# Autodesk Inventor assembly: ESP32ParasiteMicroscope_v0
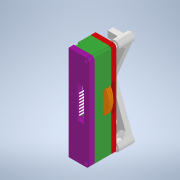
[picture p0: Inventor's stored thumbnail of the model, 180x180]
Saved by Autodesk Inventor 2022 (Build 260153000, 153)
## iProperties
Created: 2022-02-01
Part Number: ESP32ParasiteMicroscope_v0
Document SubType Name: Assembly
Designer: diederichbenedict
Author: diederichbenedict
## Documents named in this file (9)
- C:\Users\Prakash Lab\Documents\Matchboxscope\INVENTOR\ESP32ParasiteMicroscope_v0.iam
- C:\Users\Prakash Lab\Documents\Matchboxscope\INVENTOR\00_chip.ipt
- C:\Users\Prakash Lab\Documents\Matchboxscope\INVENTOR\00_ESP3-CAM.iam
- C:\Users\Prakash Lab\Documents\Matchboxscope\INVENTOR\ESP32ParasiteMicroscope_base_v0.ipt
- C:\Users\Prakash Lab\Documents\Matchboxscope\INVENTOR\ESP32ParasiteMicroscope_top_v0.ipt
- C:\Users\Prakash Lab\Documents\Matchboxscope\INVENTOR\ESP32ParasiteMicroscope_lid_v0.ipt
- C:\Users\diederichbenedict\Documents\Inventor\Content Center Files\R2022\de-DE\DIN 912\DIN 912 - M3 x 0.5 x 25 x 18.ipt
- C:\Users\Prakash Lab\Documents\Matchboxscope\INVENTOR\ESP32ParasiteMicroscope_middle_v1.ipt
- C:\Users\Prakash Lab\Documents\Matchboxscope\INVENTOR\ESP32ParasiteMicroscope_focusknob_v1.ipt
## Components (12 placed, 8 different names)
1. 00_chip:1
2. ESP32ParasiteMicroscope_base_v0:1 — Fluchtend:3, Fluchtend:4
3. ESP32ParasiteMicroscope_middle_v1:1 — Fluchtend:3, Fluchtend:4, Fluchtend:5, Fluchtend:6, Fluchtend:8, Fluchtend:9
4. ESP32ParasiteMicroscope_focusknob_v1:1 — Fluchtend:5, Fluchtend:6, Passend:1
5. ESP32ParasiteMicroscope_top_v0:1 — Fluchtend:8, Fluchtend:9, Fluchtend:10, Fluchtend:11
6. ESP32ParasiteMicroscope_lid_v0:1 — Fluchtend:10, Fluchtend:11, Einfügen:6
7. DIN 912 - ersetzt durch DIN EN ISO 4762 M3 x 25:1
8. DIN 912 - ersetzt durch DIN EN ISO 4762 M3 x 25:2
9. DIN 912 - ersetzt durch DIN EN ISO 4762 M3 x 25:3
10. DIN 912 - ersetzt durch DIN EN ISO 4762 M3 x 25:4
11. DIN 912 - ersetzt durch DIN EN ISO 4762 M3 x 25:5 — Einfügen:6
12. 00_ESP3-CAM:1 [sub-assembly] — Passend:1
## Relationships (10: Flush 8, Insert 1, Mate 1)
- Fluchtend:3 [Flush]: ESP32ParasiteMicroscope_base_v0:1 ↔ ESP32ParasiteMicroscope_middle_v1:1
- Fluchtend:4 [Flush]: ESP32ParasiteMicroscope_base_v0:1 ↔ ESP32ParasiteMicroscope_middle_v1:1
- Fluchtend:5 [Flush]: ESP32ParasiteMicroscope_middle_v1:1 ↔ ESP32ParasiteMicroscope_focusknob_v1:1
- Fluchtend:6 [Flush]: ESP32ParasiteMicroscope_middle_v1:1 ↔ ESP32ParasiteMicroscope_focusknob_v1:1
- Fluchtend:8 [Flush]: ESP32ParasiteMicroscope_middle_v1:1 ↔ ESP32ParasiteMicroscope_top_v0:1
- Fluchtend:9 [Flush]: ESP32ParasiteMicroscope_middle_v1:1 ↔ ESP32ParasiteMicroscope_top_v0:1
- Fluchtend:10 [Flush]: ESP32ParasiteMicroscope_top_v0:1 ↔ ESP32ParasiteMicroscope_lid_v0:1
- Fluchtend:11 [Flush] (15 mm): ESP32ParasiteMicroscope_top_v0:1 ↔ ESP32ParasiteMicroscope_lid_v0:1
- Einfügen:6 [Insert] (10 mm): ESP32ParasiteMicroscope_lid_v0:1 ↔ DIN 912 - ersetzt durch DIN EN ISO 4762 M3 x 25:5
- Passend:1 [Mate]: ESP32ParasiteMicroscope_focusknob_v1:1 ↔ 00_ESP3-CAM:1
